# Autodesk Inventor assembly: Assieme1
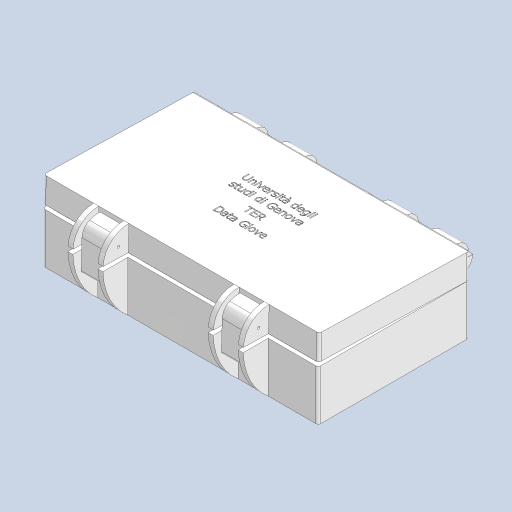
[picture p0: Inventor's stored thumbnail of the model, 512x512]
Saved by Autodesk Inventor 2023.2 (Build 272271030, 271C)
## iProperties
Created: 2023-02-08
Part Number: Assieme1
Document SubType Name: Assembly
Designer: daler
Author: daler
## Documents named in this file (10)
- C:\Users\daler\OneDrive\Desktop\Tesi Robotica\Supporti lato robot\Assieme1.iam
- C:\Users\daler\OneDrive\Desktop\Tesi Robotica\Supporti lato robot\Scatola sotto.ipt
- C:\Users\daler\OneDrive\Desktop\Tesi Robotica\Supporti lato robot\Scatola sopra.ipt
- C:\Users\daler\OneDrive\Desktop\Tesi Robotica\Supporti lato robot\Gancio1.ipt
- C:\Users\daler\OneDrive\Desktop\Tesi Robotica\Supporti lato robot\Assieme1\AIP\FEA\e8nfwvxuo.fins
- C:\Users\daler\OneDrive\Desktop\Tesi Robotica\Supporti lato robot\Assieme1\AIP\FEA\e8nfwvxuo.fsat
- C:\Users\daler\OneDrive\Desktop\Tesi Robotica\Supporti lato robot\Assieme1\AIP\FEA\e8nfwvxuo.ftes
- C:\Users\daler\OneDrive\Desktop\Tesi Robotica\Supporti lato robot\Assieme1\AIP\FEA\e8nfwvxuo.fwiz
- C:\Users\daler\OneDrive\Desktop\Tesi Robotica\Supporti lato robot\Assieme1\AIP\FEA\e8nfwvxz4.fmsh
- C:\Users\daler\OneDrive\Desktop\Tesi Robotica\Supporti lato robot\Assieme1\AIP\FEA\e8nfwvxz5.fres
## Components (4 placed, 3 different names)
1. Scatola sotto:1 — Rotazionale:1
2. Scatola sopra:1 — Rotazionale:1, Rigido:3, Rigido:4
3. Gancio1:1 — Rigido:3
4. Gancio1:2 — Rigido:4
## Relationships (3: WeldJoint 2, RevoluteJoint 1)
- Rotazionale:1 [RevoluteJoint] (1 mm): Scatola sotto:1 ↔ Scatola sopra:1
- Rigido:3 [WeldJoint]: Scatola sopra:1 ↔ Gancio1:1
- Rigido:4 [WeldJoint]: Scatola sopra:1 ↔ Gancio1:2
## Named parameters: sa_0 = 7000, sa_2 = 5000, sa_1 = 10000
note: some values were not read from the file. Shown as the stored number, unit unknown: "sa_0", "sa_2", "sa_1".
